# Autodesk Inventor assembly: драйвер
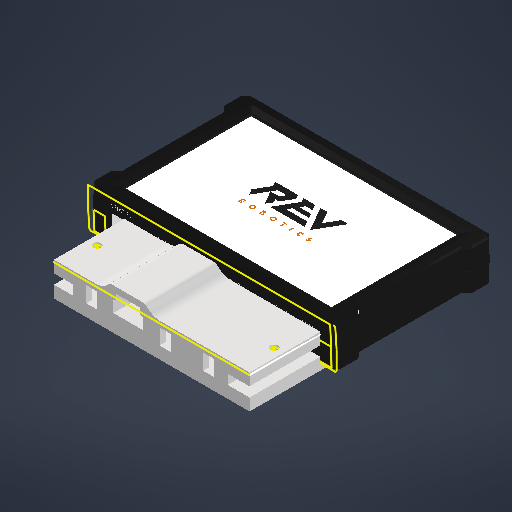
[picture p0: Inventor's stored thumbnail of the model, 512x512]
Saved by Autodesk Inventor 2025 (Build 290162000, 162)
## iProperties
Created: 2025-03-13
Part Number: драйвер
Document SubType Name: Assembly
Designer: Phantom
Author: Phantom
## Documents named in this file (4)
- C:\Users\Phantom\Desktop\Phantom16950\драйвер.iam
- C:\Users\Phantom\Downloads\REV-31-1596\REV-31-1596.ipt
- C:\Users\Phantom\Desktop\Phantom16950\драйвер.ipt
- C:\Users\Phantom\Desktop\Phantom16950\драйвер 2.ipt
## Components (3 placed, 3 different names)
1. REV-31-1596:1 — Совмещение:2, Совмещение:3
2. драйвер:1 — Совмещение:2, Совмещение:3, Совмещение:4, Совмещение:5, Заподлицо:7
3. драйвер 2:1 — Совмещение:4, Совмещение:5, Заподлицо:7
## Relationships (5: Mate 4, Flush 1)
- Совмещение:2 [Mate]: REV-31-1596:1 ↔ драйвер:1
- Совмещение:3 [Mate]: REV-31-1596:1 ↔ драйвер:1
- Совмещение:4 [Mate]: драйвер:1 ↔ драйвер 2:1
- Совмещение:5 [Mate]: драйвер:1 ↔ драйвер 2:1
- Заподлицо:7 [Flush]: драйвер:1 ↔ драйвер 2:1
